# Autodesk Inventor assembly: Assembly
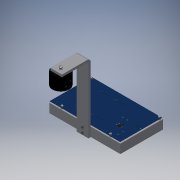
[picture p0: Inventor's stored thumbnail of the model, 180x180]
Saved by Autodesk Inventor 2017 (Build 210142000, 142)
## iProperties
Created: 2016-04-04
Part Number: Assembly
Document SubType Name: Assembly
Designer: Andres
Author: Andres
## Documents named in this file (9)
- \\Mac\Home\Documents\repositorios\MagLev\CAD\Assembly\Assembly.iam
- Z:\Documents\repositorios\MagLev\CAD\Parts\Base.ipt
- Z:\Documents\repositorios\MagLev\CAD\Parts\Brazo.ipt
- Z:\Documents\repositorios\MagLev\CAD\Parts\Coil.ipt
- \\Mac\Home\Documents\repositorios\MagLev\CAD\Assembly\Assembly\Design Accelerator\Bolted Connection3.iam
- \\Mac\Home\Documents\repositorios\MagLev\CAD\Assembly\Assembly\Design Accelerator\Bolted Connection2.iam
- Z:\Documents\repositorios\MagLev\CAD\PCB\STEP\PCB_MagLev.iam
- Z:\Documents\repositorios\MagLev\CAD\Parts\Separador.ipt
- \\Mac\Home\Documents\repositorios\MagLev\CAD\Assembly\Assembly\Design Accelerator\Bolted Connection4.iam
## Components (15 placed, 6 different names)
1. Brazo:1 — Rigid:2, Rigid:3, Mate:1, Mate:2, Rotational:1, Mate:3, Mate:4
2. Coil:1 — Rigid:2
3. Base:1 — Rigid:3, Rigid:4, Rigid:8, Rigid:10, Rigid:11, Mate:6
4. Bolted Connection:1 [sub-assembly] — Mate:1, Mate:2
5. Bolted Connection:2 [sub-assembly] — Rotational:1
6. Bolted Connection:3 [sub-assembly] — Mate:3, Mate:4
7. PCB_MagLev:1 [sub-assembly] — Rigid:9, Mate:5, Rotational:2, Rotational:3, Rotational:4
8. Separador:1 — Rigid:4
9. Separador:2 — Rigid:8, Rigid:9
10. Separador:3 — Rigid:11
11. Separador:4 — Rigid:10
12. Bolted Connection:4 [sub-assembly] — Mate:5, Mate:6
13. Bolted Connection:5 [sub-assembly] — Rotational:2
14. Bolted Connection:6 [sub-assembly] — Rotational:3
15. Bolted Connection:7 [sub-assembly] — Rotational:4
## Relationships (17: WeldJoint 7, Mate 6, RevoluteJoint 4)
- Rigid:2 [WeldJoint]: Brazo:1 ↔ Coil:1
- Rigid:3 [WeldJoint]: Brazo:1 ↔ Base:1
- Mate:1: Brazo:1 ↔ Bolted Connection:1
- Mate:2: Brazo:1 ↔ Bolted Connection:1
- Rotational:1 [RevoluteJoint]: Brazo:1 ↔ Bolted Connection:2
- Mate:3: Brazo:1 ↔ Bolted Connection:3
- Mate:4: Brazo:1 ↔ Bolted Connection:3
- Rigid:4 [WeldJoint]: Base:1 ↔ Separador:1
- Rigid:8 [WeldJoint]: Base:1 ↔ Separador:2
- Rigid:9 [WeldJoint]: PCB_MagLev:1 ↔ Separador:2
- Rigid:10 [WeldJoint]: Base:1 ↔ Separador:4
- Rigid:11 [WeldJoint]: Base:1 ↔ Separador:3
- Mate:5: PCB_MagLev:1 ↔ Bolted Connection:4
- Mate:6: Base:1 ↔ Bolted Connection:4
- Rotational:2 [RevoluteJoint]: PCB_MagLev:1 ↔ Bolted Connection:5
- Rotational:3 [RevoluteJoint]: PCB_MagLev:1 ↔ Bolted Connection:6
- Rotational:4 [RevoluteJoint]: PCB_MagLev:1 ↔ Bolted Connection:7
